# Autodesk Inventor assembly: updated table+legs
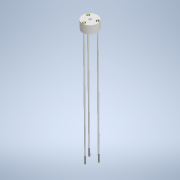
[picture p0: Inventor's stored thumbnail of the model, 180x180]
Saved by Autodesk Inventor 2020 (Build 240168000, 168)
## iProperties
Created: 2019-06-14
Part Number: updated table+legs
Document SubType Name: Assembly
Designer: ColinP
Author: ColinP
## Documents named in this file (6)
- C:\Users\ColinP\Documents\Inventor\igor\updated table+legs.iam
- C:\Users\ColinP\Documents\Inventor\igor\table.ipt
- C:\Users\ColinP\Documents\Inventor\igor\eyelet.ipt
- C:\Users\ColinP\Documents\Inventor\igor\assembly of 13 and 2.iam
- C:\Users\ColinP\Documents\Inventor\igor\washer.ipt
- C:\Users\ColinP\Documents\Inventor\Content Center Files\R2020\en-US\ISO 4036(2)\ISO 4036 - M3(2).ipt
## Components (16 placed, 5 different names)
1. table:1 — Insert:1, Insert:3, Insert:4, Insert:5, Insert:8, Insert:9, Insert:10, Insert:11
2. eyelet:1 — Insert:1, Insert:13
3. eyelet:2 — Insert:9
4. eyelet:3 — Insert:5, Insert:12
5. eyelet:4 — Insert:3, Insert:14
6. eyelet:6 — Insert:4, Insert:11
7. eyelet:7 — Insert:8, Insert:10
8. assembly of 13 and 2:1 [sub-assembly] — Insert:13, Insert:15
9. assembly of 13 and 2:2 [sub-assembly] — Insert:12, Insert:16, Insert:20
10. assembly of 13 and 2:3 [sub-assembly] — Insert:14, Insert:17, Insert:19
11. washer:1 — Insert:15, Insert:18
12. washer:2 — Insert:16
13. washer:3 — Insert:17
14. ISO 4036 M3:1 — Insert:18
15. ISO 4036 M3:2 — Insert:20
16. ISO 4036 M3:3 — Insert:19
## Relationships (17: Insert 17)
- Insert:1: table:1 ↔ eyelet:1
- Insert:3: table:1 ↔ eyelet:4
- Insert:4: table:1 ↔ eyelet:6
- Insert:5: table:1 ↔ eyelet:3
- Insert:8: table:1 ↔ eyelet:7
- Insert:9: table:1 ↔ eyelet:2
- Insert:10: table:1 ↔ eyelet:7
- Insert:11: table:1 ↔ eyelet:6
- Insert:12 (-4.064 mm): eyelet:3 ↔ assembly of 13 and 2:2
- Insert:13 (-4.064 mm): eyelet:1 ↔ assembly of 13 and 2:1
- Insert:14 (-4.064 mm): eyelet:4 ↔ assembly of 13 and 2:3
- Insert:15 (-2.286 mm): assembly of 13 and 2:1 ↔ washer:1
- Insert:16 (-2.286 mm): assembly of 13 and 2:2 ↔ washer:2
- Insert:17 (-2.286 mm): assembly of 13 and 2:3 ↔ washer:3
- Insert:18: washer:1 ↔ ISO 4036 M3:1
- Insert:19: assembly of 13 and 2:3 ↔ ISO 4036 M3:3
- Insert:20 (-0.254 mm): assembly of 13 and 2:2 ↔ ISO 4036 M3:2
